# Autodesk Inventor assembly: タミヤダンパー
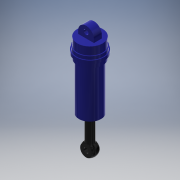
[picture p0: Inventor's stored thumbnail of the model, 180x180]
Saved by Autodesk Inventor 2017 (Build 210142000, 142)
## iProperties
Part Number: タミヤダンパー
Material: 一般
Document SubType Name: Assembly
Designer: 雪村
Mass: 27 g
Surface Area: 42.7382 cm^2
Volume: 8.21829 cm^3
Density: 3.28536 g/cm^3
Author: 雪村
## Documents named in this file (3)
- C:\Users\white\OneDrive\ドキュメント\Inventor_2017\2018年機体\2018年2年機体　雪村\タミヤダンパー.iam
- C:\Users\white\OneDrive\ドキュメント\Inventor_2017\2018年機体\2018年2年機体　雪村\タミヤダンパー.ipt
- C:\Users\white\OneDrive\ドキュメント\Inventor_2017\2018年機体\2018年2年機体　雪村\タミヤダンパー、シャフト.ipt
## Components (2 placed, 2 different names)
1. タミヤダンパー:1 — メイト:1, フラッシュ:1
2. タミヤダンパー、シャフト:1 — メイト:1, フラッシュ:1
## Relationships (2: Mate 1, Flush 1)
- メイト:1 [Mate]: タミヤダンパー:1 ↔ タミヤダンパー、シャフト:1
- フラッシュ:1 [Flush]: タミヤダンパー:1 ↔ タミヤダンパー、シャフト:1
